# Autodesk Inventor assembly: Gestell_zsm
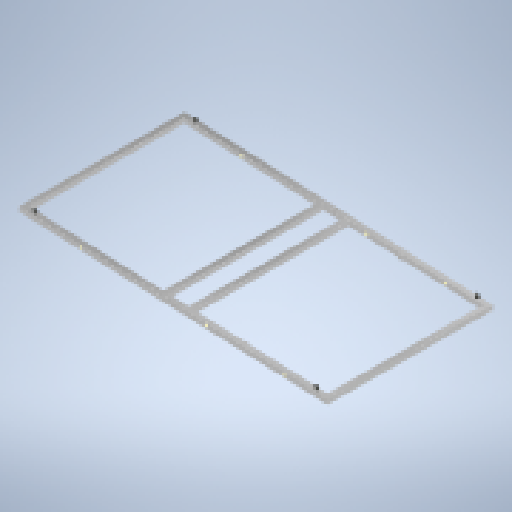
[picture p0: Inventor's stored thumbnail of the model, 512x512]
Saved by Autodesk Inventor 2024.4 (Build 284460000, 460)
## iProperties
Created: 2026-01-11
Part Number: Gestell_zsm
Description: Gestell_zsm
Document SubType Name: Assembly
Designer: julia
Mass: 8962.49 g
Surface Area: 31235.3 cm^2
Volume: 3255.62 cm^3
Density: 2.75293 g/cm^3
DocNumber: Gestell_zsm.iam
Folder: I60-Konstruktion\I60-Gruppe-7\Gestell\
VDS_Category: Konstruktion
Masse[kg]: 8,962 kg
## Documents named in this file (9)
- C:\Users\Philf\Documents\Vault\Daten\I60-Konstruktion\I60-Gruppe-7\Gestell\Gestell_zsm.iam
- C:\Users\Philf\Documents\Vault\Daten\I60-Konstruktion\I60-Gruppe-7\Gestell\Verbinder.ipt
- C:\Users\Philf\Documents\Vault\Daten\I60-Konstruktion\I60-Gruppe-7\Gestell\Längs_Traverse_hinten.ipt
- C:\Users\Philf\Documents\Vault\Daten\I60-Konstruktion\I60-Gruppe-7\Gestell\Längs_Traverse_vorne.ipt
- C:\Users\Philf\Documents\Vault\Daten\I60-Konstruktion\I60-Gruppe-7\Gestell\Ouertraverse_vorne.ipt
- C:\Users\Philf\Documents\Vault\Daten\I60-Konstruktion\I60-Gruppe-7\Gestell\Quer_Traverse_Sitz.ipt
- C:\Users\Philf\Documents\Vault\Daten\I60-Konstruktion\I60-Gruppe-7\Gestell\Traversen_Deckel.ipt
- C:\Users\Philf\Documents\Vault\Daten\I60-Konstruktion\I60-Gruppe-7\Gestell\Lager_Schaufelrad.ipt
- C:\Users\Philf\Documents\Vault\Daten\I60-Konstruktion\I60-Gruppe-7\Gestell\3112T51_Zinc-Plated Steel Round Eye Nut - for Lifting.ipt
## Components (30 placed, 8 different names)
1. Verbinder:1 — Passend:67, Passend:68, Passend:69
2. Verbinder:2 — Passend:61, Passend:62, Passend:63, Passend:64, Passend:65, Passend:66
3. Längs_Traverse_hinten:1 — Passend:35, Fluchtend:17, Passend:43, Passend:44, Passend:49, Passend:50, Winkel:2, Passend:57, Passend:64, Passend:65, Passend:66, Passend:70, Fluchtend:21, Fluchtend:22
4. Längs_Traverse_hinten:2 — Fluchtend:15, Passend:34, Fluchtend:16, Passend:36, Fluchtend:18, Passend:45, Passend:46, Passend:51, Passend:52, Winkel:3, Passend:67, Passend:68, Passend:69
5. Längs_Traverse_vorne:1 — Fluchtend:7, Fluchtend:8, Passend:38, Fluchtend:20, Passend:41, Passend:42, Passend:47, Passend:48, Winkel:1, Passend:60, Passend:61, Passend:62, Passend:63, Passend:73, Fluchtend:24, Passend:76, Passend:77, Winkel:6
6. Längs_Traverse_vorne:2 — Fluchtend:9, Fluchtend:10, Passend:26, Passend:37, Fluchtend:19, Passend:39, Passend:40, Passend:53, Passend:54, Winkel:4, Passend:71, Fluchtend:23, Passend:74, Passend:75, Winkel:5
7. Quer_Traverse_Sitz:1 — Passend:58, Passend:59, Passend:60
8. Quer_Traverse_Sitz:2 — Passend:55, Passend:56, Passend:57
9. Traversen_Deckel:1 — Passend:51, Passend:52, Winkel:3
10. Traversen_Deckel:2 — Passend:22, Fluchtend:5, Passend:23
11. Traversen_Deckel:3 — Passend:53, Passend:54, Winkel:4
12. Traversen_Deckel:4 — Passend:47, Passend:48, Winkel:1, Passend:58, Passend:59
13. Traversen_Deckel:5 — Passend:49, Passend:50, Winkel:2, Passend:55, Passend:56
14. Traversen_Deckel:6 — Passend:24, Fluchtend:6, Passend:25
15. Ouertraverse_vorne:1 — Passend:22, Fluchtend:5, Passend:23, Passend:24, Fluchtend:6, Passend:25, Fluchtend:7, Fluchtend:8, Fluchtend:9, Fluchtend:10, Passend:26
16. Traversen_Deckel:7 — Fluchtend:13, Passend:29, Passend:30
17. Traversen_Deckel:8 — Passend:32, Passend:33, Fluchtend:14, Passend:70
18. Ouertraverse_vorne:2 — Fluchtend:13, Passend:29, Passend:30, Passend:32, Passend:33, Fluchtend:14, Fluchtend:15, Passend:34, Fluchtend:16, Fluchtend:21, Fluchtend:22
19. Lager_Schaufelrad:1 — Passend:36, Fluchtend:18
20. Lager_Schaufelrad:2 — Passend:35, Fluchtend:17
21. Lager_Schaufelrad:3 — Passend:38, Fluchtend:20
22. Lager_Schaufelrad:4 — Passend:37, Fluchtend:19
23. 3112T51_Zinc-Plated Steel Round Eye Nut - for Lifting:1 — Passend:39, Passend:40
24. 3112T51_Zinc-Plated Steel Round Eye Nut - for Lifting:2 — Passend:41, Passend:42
25. 3112T51_Zinc-Plated Steel Round Eye Nut - for Lifting:3 — Passend:45, Passend:46
26. 3112T51_Zinc-Plated Steel Round Eye Nut - for Lifting:4 — Passend:43, Passend:44
27. Lager_Schaufelrad:5 — Passend:73, Fluchtend:24
28. Lager_Schaufelrad:6 — Passend:71, Fluchtend:23
29. Traversen_Deckel:9 — Passend:76, Passend:77, Winkel:6
30. Traversen_Deckel:10 — Passend:74, Passend:75, Winkel:5
## Relationships (76: Mate 52, Flush 18, Angle 6)
- Passend:22 [Mate]: Traversen_Deckel:2 ↔ Ouertraverse_vorne:1
- Fluchtend:5 [Flush]: Traversen_Deckel:2 ↔ Ouertraverse_vorne:1
- Passend:23 [Mate]: Traversen_Deckel:2 ↔ Ouertraverse_vorne:1
- Passend:24 [Mate]: Traversen_Deckel:6 ↔ Ouertraverse_vorne:1
- Fluchtend:6 [Flush]: Traversen_Deckel:6 ↔ Ouertraverse_vorne:1
- Passend:25 [Mate]: Traversen_Deckel:6 ↔ Ouertraverse_vorne:1
- Fluchtend:7 [Flush]: Längs_Traverse_vorne:1 ↔ Ouertraverse_vorne:1
- Fluchtend:8 [Flush]: Längs_Traverse_vorne:1 ↔ Ouertraverse_vorne:1
- Fluchtend:9 [Flush]: Längs_Traverse_vorne:2 ↔ Ouertraverse_vorne:1
- Fluchtend:10 [Flush]: Längs_Traverse_vorne:2 ↔ Ouertraverse_vorne:1
- Passend:26 [Mate]: Längs_Traverse_vorne:2 ↔ Ouertraverse_vorne:1
- Fluchtend:13 [Flush]: Traversen_Deckel:7 ↔ Ouertraverse_vorne:2
- Passend:29 [Mate]: Traversen_Deckel:7 ↔ Ouertraverse_vorne:2
- Passend:30 [Mate]: Traversen_Deckel:7 ↔ Ouertraverse_vorne:2
- Passend:32 [Mate]: Traversen_Deckel:8 ↔ Ouertraverse_vorne:2
- Passend:33 [Mate]: Traversen_Deckel:8 ↔ Ouertraverse_vorne:2
- Fluchtend:14 [Flush]: Traversen_Deckel:8 ↔ Ouertraverse_vorne:2
- Fluchtend:15 [Flush]: Längs_Traverse_hinten:2 ↔ Ouertraverse_vorne:2
- Passend:34 [Mate]: Längs_Traverse_hinten:2 ↔ Ouertraverse_vorne:2
- Fluchtend:16 [Flush]: Längs_Traverse_hinten:2 ↔ Ouertraverse_vorne:2
- Passend:35 [Mate]: Längs_Traverse_hinten:1 ↔ Lager_Schaufelrad:2
- Fluchtend:17 [Flush]: Längs_Traverse_hinten:1 ↔ Lager_Schaufelrad:2
- Passend:36 [Mate]: Längs_Traverse_hinten:2 ↔ Lager_Schaufelrad:1
- Fluchtend:18 [Flush]: Längs_Traverse_hinten:2 ↔ Lager_Schaufelrad:1
- Passend:37 [Mate]: Längs_Traverse_vorne:2 ↔ Lager_Schaufelrad:4
- Fluchtend:19 [Flush]: Längs_Traverse_vorne:2 ↔ Lager_Schaufelrad:4
- Passend:38 [Mate]: Längs_Traverse_vorne:1 ↔ Lager_Schaufelrad:3
- Fluchtend:20 [Flush]: Längs_Traverse_vorne:1 ↔ Lager_Schaufelrad:3
- Passend:39 [Mate]: Längs_Traverse_vorne:2 ↔ 3112T51_Zinc-Plated Steel Round Eye Nut - for Lifting:1
- Passend:40 [Mate]: Längs_Traverse_vorne:2 ↔ 3112T51_Zinc-Plated Steel Round Eye Nut - for Lifting:1
- Passend:41 [Mate]: Längs_Traverse_vorne:1 ↔ 3112T51_Zinc-Plated Steel Round Eye Nut - for Lifting:2
- Passend:42 [Mate]: Längs_Traverse_vorne:1 ↔ 3112T51_Zinc-Plated Steel Round Eye Nut - for Lifting:2
- Passend:43 [Mate]: Längs_Traverse_hinten:1 ↔ 3112T51_Zinc-Plated Steel Round Eye Nut - for Lifting:4
- Passend:44 [Mate]: Längs_Traverse_hinten:1 ↔ 3112T51_Zinc-Plated Steel Round Eye Nut - for Lifting:4
- Passend:45 [Mate]: Längs_Traverse_hinten:2 ↔ 3112T51_Zinc-Plated Steel Round Eye Nut - for Lifting:3
- Passend:46 [Mate]: Längs_Traverse_hinten:2 ↔ 3112T51_Zinc-Plated Steel Round Eye Nut - for Lifting:3
- Passend:47 [Mate]: Längs_Traverse_vorne:1 ↔ Traversen_Deckel:4
- Passend:48 [Mate]: Längs_Traverse_vorne:1 ↔ Traversen_Deckel:4
- Winkel:1 [Angle] (0 deg): Längs_Traverse_vorne:1 ↔ Traversen_Deckel:4
- Passend:49 [Mate]: Längs_Traverse_hinten:1 ↔ Traversen_Deckel:5
- Passend:50 [Mate]: Längs_Traverse_hinten:1 ↔ Traversen_Deckel:5
- Winkel:2 [Angle] (0 deg): Längs_Traverse_hinten:1 ↔ Traversen_Deckel:5
- Passend:51 [Mate]: Längs_Traverse_hinten:2 ↔ Traversen_Deckel:1
- Passend:52 [Mate]: Längs_Traverse_hinten:2 ↔ Traversen_Deckel:1
- Winkel:3 [Angle] (0 deg): Längs_Traverse_hinten:2 ↔ Traversen_Deckel:1
- Passend:53 [Mate]: Längs_Traverse_vorne:2 ↔ Traversen_Deckel:3
- Passend:54 [Mate]: Längs_Traverse_vorne:2 ↔ Traversen_Deckel:3
- Winkel:4 [Angle] (0 deg): Längs_Traverse_vorne:2 ↔ Traversen_Deckel:3
- Passend:55 [Mate]: Quer_Traverse_Sitz:2 ↔ Traversen_Deckel:5
- Passend:56 [Mate]: Quer_Traverse_Sitz:2 ↔ Traversen_Deckel:5
- Passend:57 [Mate]: Längs_Traverse_hinten:1 ↔ Quer_Traverse_Sitz:2
- Passend:58 [Mate]: Quer_Traverse_Sitz:1 ↔ Traversen_Deckel:4
- Passend:59 [Mate]: Quer_Traverse_Sitz:1 ↔ Traversen_Deckel:4
- Passend:60 [Mate]: Längs_Traverse_vorne:1 ↔ Quer_Traverse_Sitz:1
- Passend:61 [Mate]: Verbinder:2 ↔ Längs_Traverse_vorne:1
- Passend:62 [Mate]: Verbinder:2 ↔ Längs_Traverse_vorne:1
- Passend:63 [Mate]: Verbinder:2 ↔ Längs_Traverse_vorne:1
- Passend:64 [Mate]: Verbinder:2 ↔ Längs_Traverse_hinten:1
- Passend:65 [Mate]: Verbinder:2 ↔ Längs_Traverse_hinten:1
- Passend:66 [Mate]: Verbinder:2 ↔ Längs_Traverse_hinten:1
- Passend:67 [Mate]: Verbinder:1 ↔ Längs_Traverse_hinten:2
- Passend:68 [Mate]: Verbinder:1 ↔ Längs_Traverse_hinten:2
- Passend:69 [Mate]: Verbinder:1 ↔ Längs_Traverse_hinten:2
- Passend:70 [Mate]: Längs_Traverse_hinten:1 ↔ Traversen_Deckel:8
- Fluchtend:21 [Flush]: Längs_Traverse_hinten:1 ↔ Ouertraverse_vorne:2
- Fluchtend:22 [Flush]: Längs_Traverse_hinten:1 ↔ Ouertraverse_vorne:2
- Passend:71 [Mate]: Längs_Traverse_vorne:2 ↔ Lager_Schaufelrad:6
- Fluchtend:23 [Flush]: Längs_Traverse_vorne:2 ↔ Lager_Schaufelrad:6
- Passend:73 [Mate]: Längs_Traverse_vorne:1 ↔ Lager_Schaufelrad:5
- Fluchtend:24 [Flush]: Längs_Traverse_vorne:1 ↔ Lager_Schaufelrad:5
- Passend:74 [Mate]: Längs_Traverse_vorne:2 ↔ Traversen_Deckel:10
- Passend:75 [Mate]: Längs_Traverse_vorne:2 ↔ Traversen_Deckel:10
- Winkel:5 [Angle] (0 deg): Längs_Traverse_vorne:2 ↔ Traversen_Deckel:10
- Passend:76 [Mate]: Längs_Traverse_vorne:1 ↔ Traversen_Deckel:9
- Passend:77 [Mate]: Längs_Traverse_vorne:1 ↔ Traversen_Deckel:9
- Winkel:6 [Angle] (0 deg): Längs_Traverse_vorne:1 ↔ Traversen_Deckel:9
